# Autodesk Inventor assembly: Assembly1
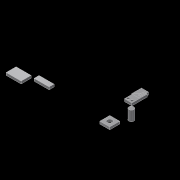
[picture p0: Inventor's stored thumbnail of the model, 180x180]
Saved by Autodesk Inventor 2021.1 (Build 251245000, 245)
## iProperties
RuleStatus: InUse
Created: 2020-08-31
Part Number: Assembly1
Document SubType Name: Assembly
Designer: Hashimoto
Author: Hashimoto
## Documents named in this file (7)
- Z:\inventorroom\cad\Assembly1.iam
- Z:\inventorroom\cad\Part1.ipt
- Z:\inventorroom\cad\Part2.ipt
- Z:\inventorroom\cad\Part3.ipt
- Z:\inventorroom\cad\Part4.ipt
- Z:\inventorroom\cad\Part5.ipt
- Z:\inventorroom\cad\Part6.ipt
## Components (6 placed, 6 different names)
1. Part1:1 — フラッシュ:1
2. Part2:1 — フラッシュ:1
3. Part3:1
4. Part4:1
5. Part5:1
6. Part6:1
## Relationships (1: Flush 1)
- フラッシュ:1 [Flush]: Part1:1 ↔ Part2:1
